# Autodesk Inventor assembly: frame
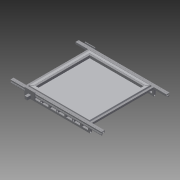
[picture p0: Inventor's stored thumbnail of the model, 180x180]
Saved by Autodesk Inventor 2013 (Build 170138000, 138)
## iProperties
Created: 2012-10-19
Part Number: frame
Document SubType Name: Assembly
Designer: Istvan
Author: Istvan
## Documents named in this file (9)
- D:\GitHub\Crown-Fire\CAD\Frame\frame.iam
- D:\GitHub\Crown-Fire\CAD\Frame\Table\table.iam
- D:\GitHub\Crown-Fire\CAD\Frame\Supports\supports.iam
- D:\GitHub\Crown-Fire\CAD\Frame\WorkTable\workTable.ipt
- D:\GitHub\Crown-Fire\CAD\Frame\GantryMount\rack.ipt
- D:\GitHub\Crown-Fire\CAD\Frame\GantryMount\cChannel.ipt
- C:\Users\istvan.burbank\Documents\GitHub\Crown-Fire\CAD\Templates\cChannel2x1.ipt
- D:\GitHub\Crown-Fire\CAD\Frame\GantryMount\vee-track.ipt
- D:\GitHub\Crown-Fire\CAD\Frame\GantryMount\tractor.iam
## Components (11 placed, 7 different names)
1. table:1 [sub-assembly] — Mate:1, Mate:2, Mate:5, Mate:6
2. supports:1 [sub-assembly] — Mate:1, Mate:2, Mate:3, Mate:4, Mate:5, Mate:6, Mate:7, Mate:8, Flush:1, Flush:2, Flush:3, Flush:4
3. workTable:1 — Mate:3, Mate:4
4. rack:1 — Flush:5, Mate:15
5. rack:2 — Flush:6, Mate:14
6. cChannel:1 — Mate:8, Flush:2, Flush:4, Flush:5, Mate:11, Flush:8, Mate:15, Mate:17
7. cChannel:2 — Mate:7, Flush:1, Flush:3, Flush:6, Mate:12, Flush:7, Mate:14, Mate:16
8. vee-track:1 — Mate:12, Flush:7, Tangent:1, Tangent:2, Tangent:6, Mate:16
9. vee-track:2 — Mate:11, Flush:8, Mate:17, Tangent:7, Tangent:8, Tangent:9
10. tractor:1 [sub-assembly] — Tangent:1, Tangent:2, Tangent:6
11. tractor:2 [sub-assembly] — Tangent:7, Tangent:8, Tangent:9
## Relationships (28: Mate 14, Flush 8, Tangent 6)
- Mate:1 (12.7 mm): table:1 ↔ supports:1
- Mate:2 (12.7 mm): table:1 ↔ supports:1
- Mate:3: supports:1 ↔ workTable:1
- Mate:4: supports:1 ↔ workTable:1
- Mate:5: table:1 ↔ supports:1
- Mate:6 (6.35 mm): table:1 ↔ supports:1
- Mate:7: supports:1 ↔ cChannel:2
- Mate:8: supports:1 ↔ cChannel:1
- Flush:1: supports:1 ↔ cChannel:2
- Flush:2: supports:1 ↔ cChannel:1
- Flush:3: supports:1 ↔ cChannel:2
- Flush:4: supports:1 ↔ cChannel:1
- Flush:5: rack:1 ↔ cChannel:1
- Flush:6: rack:2 ↔ cChannel:2
- Mate:11: cChannel:1 ↔ vee-track:2
- Mate:12: cChannel:2 ↔ vee-track:1
- Flush:7: cChannel:2 ↔ vee-track:1
- Flush:8: cChannel:1 ↔ vee-track:2
- Mate:14: rack:2 ↔ cChannel:2
- Mate:15: rack:1 ↔ cChannel:1
- Tangent:1: vee-track:1 ↔ tractor:1
- Tangent:2: vee-track:1 ↔ tractor:1
- Tangent:6: vee-track:1 ↔ tractor:1
- Mate:16 (12.7 mm): cChannel:2 ↔ vee-track:1
- Mate:17 (12.7 mm): cChannel:1 ↔ vee-track:2
- Tangent:7: vee-track:2 ↔ tractor:2
- Tangent:8: vee-track:2 ↔ tractor:2
- Tangent:9: vee-track:2 ↔ tractor:2
